# Autodesk Inventor assembly: TR2 Arm
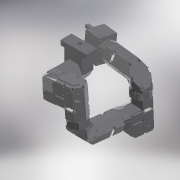
[picture p0: Inventor's stored thumbnail of the model, 180x180]
Saved by Autodesk Inventor 2017 (Build 210142000, 142)
## iProperties
Created: 2018-10-11
Part Number: TR2 Arm
Document SubType Name: Assembly
Designer: Zach
Author: Zach
## Documents named in this file (8)
- C:\Users\Dell\Documents\GitHub\tr2\Arm\Arm.iam
- C:\Users\Dell\Documents\GitHub\tr2\Arm Actuator\Arm Actuator.iam
- C:\Users\Dell\Documents\GitHub\tr2\Gripper\Gripper.iam
- C:\Users\Dell\Documents\GitHub\tr2\Arm\TARM09b.ipt
- C:\Users\Dell\Documents\GitHub\tr2\Arm\TARM01b.ipt
- C:\Users\Dell\Documents\GitHub\tr2\Arm\TARM02b.ipt
- C:\Users\Dell\Documents\GitHub\tr2\Arm\TARM14.ipt
- C:\Users\Dell\Documents\GitHub\tr2\Actuator 1.2\Actuator 1.2.iam
## Components (13 placed, 7 different names)
1. TARM01b:1 — Mate:181, Mate:182, Mate:183
2. Arm Actuator:1 [sub-assembly] — Mate:181, Mate:182, Mate:183, Mate:184, Mate:185
3. Arm Actuator:2 [sub-assembly] — Mate:173, Mate:174, Mate:175, Mate:219
4. Gripper:1 [sub-assembly] — Mate:239, Mate:240
5. TARM09b:1 — Mate:173, Mate:174, Mate:175, Mate:186, Mate:187, Mate:188, Mate:221, Mate:222, Mate:223
6. TARM09b:2 — Mate:229, Mate:230, Mate:231, Mate:232, Mate:233
7. TARM02b:1 — Mate:184, Mate:185, Mate:186, Mate:187, Mate:188
8. TARM14:1 — Mate:219, Mate:224, Mate:225, Mate:226, Mate:227, Mate:228
9. TARM14:2 — Mate:234, Mate:235, Mate:236, Mate:237, Mate:238
10. Actuator 1.2:1 [sub-assembly] — Mate:221, Mate:222, Mate:223, Mate:224, Mate:225
11. Actuator 1.2:2 [sub-assembly] — Mate:226, Mate:227, Mate:228, Mate:229, Mate:230
12. Actuator 1.2:3 [sub-assembly] — Mate:231, Mate:232, Mate:233, Mate:234, Mate:235
13. Actuator 1.2:4 [sub-assembly] — Mate:236, Mate:237, Mate:238, Mate:239, Mate:240
## Relationships (32: Mate 32)
- Mate:173: Arm Actuator:2 ↔ TARM09b:1
- Mate:174: Arm Actuator:2 ↔ TARM09b:1
- Mate:175: Arm Actuator:2 ↔ TARM09b:1
- Mate:181: TARM01b:1 ↔ Arm Actuator:1
- Mate:182: TARM01b:1 ↔ Arm Actuator:1
- Mate:183: TARM01b:1 ↔ Arm Actuator:1
- Mate:184: Arm Actuator:1 ↔ TARM02b:1
- Mate:185: Arm Actuator:1 ↔ TARM02b:1
- Mate:186: TARM09b:1 ↔ TARM02b:1
- Mate:187: TARM09b:1 ↔ TARM02b:1
- Mate:188: TARM09b:1 ↔ TARM02b:1
- Mate:219: Arm Actuator:2 ↔ TARM14:1
- Mate:221: TARM09b:1 ↔ Actuator 1.2:1
- Mate:222: TARM09b:1 ↔ Actuator 1.2:1
- Mate:223: TARM09b:1 ↔ Actuator 1.2:1
- Mate:224: TARM14:1 ↔ Actuator 1.2:1
- Mate:225: TARM14:1 ↔ Actuator 1.2:1
- Mate:226: TARM14:1 ↔ Actuator 1.2:2
- Mate:227: TARM14:1 ↔ Actuator 1.2:2
- Mate:228: TARM14:1 ↔ Actuator 1.2:2
- Mate:229: TARM09b:2 ↔ Actuator 1.2:2
- Mate:230: TARM09b:2 ↔ Actuator 1.2:2
- Mate:231: TARM09b:2 ↔ Actuator 1.2:3
- Mate:232: TARM09b:2 ↔ Actuator 1.2:3
- Mate:233: TARM09b:2 ↔ Actuator 1.2:3
- Mate:234: TARM14:2 ↔ Actuator 1.2:3
- Mate:235: TARM14:2 ↔ Actuator 1.2:3
- Mate:236: TARM14:2 ↔ Actuator 1.2:4
- Mate:237: TARM14:2 ↔ Actuator 1.2:4
- Mate:238: TARM14:2 ↔ Actuator 1.2:4
- Mate:239: Gripper:1 ↔ Actuator 1.2:4
- Mate:240: Gripper:1 ↔ Actuator 1.2:4
